# Autodesk Inventor assembly: Gripper New
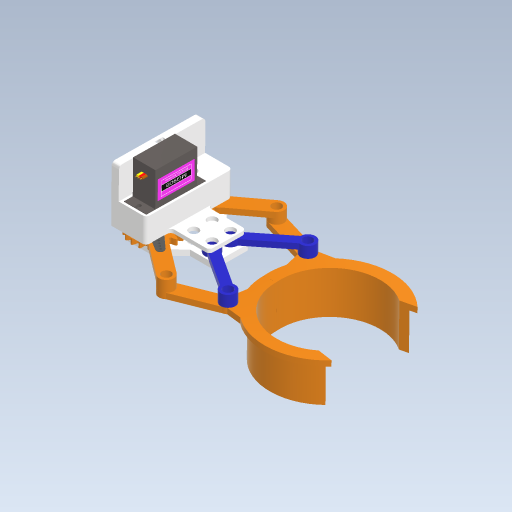
[picture p0: Inventor's stored thumbnail of the model, 512x512]
Saved by Autodesk Inventor 2023.5 (Build 275446000, 446)
## iProperties
Created: 2025-10-05
Part Number: Gripper New
Document SubType Name: Assembly
Designer: Guntur
Author: Guntur
## iProperties of the stored document MG90S_arm01.ipt
Created: 2024-09-02
Part Number: levier_servo
Material: Generic
Description: FreeCAD Model
Document SubType Name: Modeling
Designer: Guntur
Authority: Unknown
Density: 1 g/cm^3
Appearance: Default
Title: Open CASCADE Shape Model
Sending System: FreeCAD
Preprocessor: Open CASCADE STEP processor 7.6
## Documents named in this file (11)
- **F:\EEJ2025\design\Gripper New\Gripper New.iam*LocalDocs*xAaaaalcaAaaaaaaaAaaaqcdoTc*MG90S_arm01.ipt
- F:\EEJ2025\design\Gripper New\Gripper New.iam
- F:\EEJ2025\design\Gripper New\Base.ipt
- F:\EEJ2025\design\Gripper New\Gear Link.ipt
- F:\EEJ2025\design\Gripper New\Arm Link.ipt
- F:\EEJ2025\design\Gripper New\Left Hand.ipt
- F:\EEJ2025\design\Gripper New\Right Hand.ipt
- F:\backup\inv\asset\mg90s-micro-servo-2.snapshot.3\M90S_ali\M90S_ali.iam
- F:\EEJ2025\design\Gripper New\Bracket Servo.ipt
- F:\EEJ2025\design\Gripper New\Gear Link Servo.ipt
- F:\EEJ2025\design\MG90S\MG90S_arm01.step
## Components (10 placed, 9 different names)
1. Gear Link:2 — Mate:23, Mate:26, Mate:36, Mate:37, Mate:42, Mate:43
2. Arm Link:1 — Mate:24, Mate:25, Mate:40
3. Arm Link:2 — Mate:28, Mate:41
4. Right Hand:1 — Mate:23, Mate:24, Mate:25, Mate:26
5. Left Hand:1 — Mate:28, Mate:49, Mate:50
6. M90S_ali:1 [sub-assembly] — Mate:31, Mate:32, Mate:33, Mate:34, Mate:44, Mate:45
7. Bracket Servo:1 — Mate:31, Mate:32, Mate:33, Mate:34, Mate:42, Mate:43, Mate:47
8. Base:1 — Mate:36, Mate:37, Mate:40, Mate:41
9. MG90S_arm01:1 — Mate:44, Mate:45, Mate:46, Mate:48
10. Gear Link Servo:1 — Mate:46, Mate:47, Mate:48, Mate:49, Mate:50
## Relationships (22: Mate 22)
- Mate:23: Gear Link:2 ↔ Right Hand:1
- Mate:24: Arm Link:1 ↔ Right Hand:1
- Mate:25: Arm Link:1 ↔ Right Hand:1
- Mate:26: Gear Link:2 ↔ Right Hand:1
- Mate:28: Arm Link:2 ↔ Left Hand:1
- Mate:31: M90S_ali:1 ↔ Bracket Servo:1
- Mate:32: M90S_ali:1 ↔ Bracket Servo:1
- Mate:33: M90S_ali:1 ↔ Bracket Servo:1
- Mate:34: M90S_ali:1 ↔ Bracket Servo:1
- Mate:36: Gear Link:2 ↔ Base:1
- Mate:37: Gear Link:2 ↔ Base:1
- Mate:40: Arm Link:1 ↔ Base:1
- Mate:41: Arm Link:2 ↔ Base:1
- Mate:42: Gear Link:2 ↔ Bracket Servo:1
- Mate:43: Gear Link:2 ↔ Bracket Servo:1
- Mate:44: M90S_ali:1 ↔ MG90S_arm01:1
- Mate:45: M90S_ali:1 ↔ MG90S_arm01:1
- Mate:46: MG90S_arm01:1 ↔ Gear Link Servo:1
- Mate:47: Bracket Servo:1 ↔ Gear Link Servo:1
- Mate:48: MG90S_arm01:1 ↔ Gear Link Servo:1
- Mate:49: Left Hand:1 ↔ Gear Link Servo:1
- Mate:50: Left Hand:1 ↔ Gear Link Servo:1
